# Autodesk Inventor assembly: Crossbrace
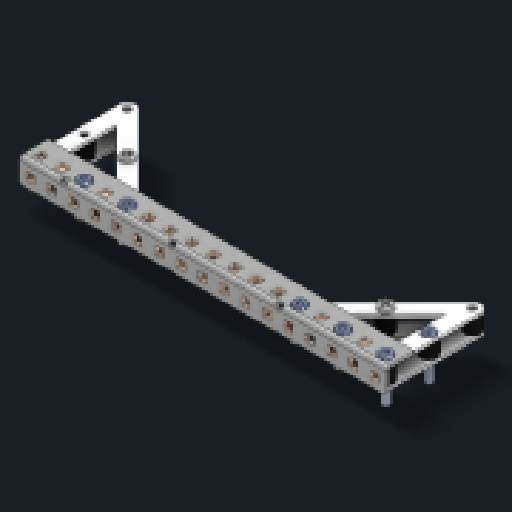
[picture p0: Inventor's stored thumbnail of the model, 512x512]
Saved by Autodesk Inventor 2025.1 (Build 291241000, 241)
## iProperties
Created: 2024-11-17
Part Number: Crossbrace
Document SubType Name: Assembly
Designer: avere
Author: avere
## Documents named in this file (14)
- C:\Users\avere\VEX\High Stakes\CAD\V3\Intake\Floating Stage\Crossbrace.iam
- C:\Users\avere\VEX\High Stakes\CAD\ROBOPROS-CAD-Inventor\Structure\C Channel\Aluminum 1x3x1 Half Thick Cut\Alu C Half Thick 1x3x1x17.ipt
- C:\Users\avere\VEX\High Stakes\CAD\V3\Intake\Floating Stage\Custom Parts\Arm Triangle Gusset.ipt
- C:\Users\avere\VEX\High Stakes\CAD\ROBOPROS-CAD-Inventor\Motion\Spacers\Spacer Nylon .375 OD.ipt
- C:\Users\avere\VEX\High Stakes\CAD\ROBOPROS-CAD-Inventor\Motion\Spacers\Spacer Nylon .375 OD\NSpacer .375 OD x .375.ipt
- C:\Users\avere\VEX\High Stakes\CAD\ROBOPROS-CAD-Inventor\Structure\Hardware\Screw Nylon - Pan Head\NScrew Pan Head Threaded .625.ipt
- C:\Users\avere\VEX\High Stakes\CAD\ROBOPROS-CAD-Inventor\Structure\Hardware\Screw Steel - Star.ipt
- C:\Users\avere\VEX\High Stakes\CAD\ROBOPROS-CAD-Inventor\Structure\Hardware\Nut Nylon\Nut Nylon - White.ipt
- C:\Users\avere\VEX\High Stakes\CAD\ROBOPROS-CAD-Inventor\Structure\Hardware\Nut Nylon.ipt
- C:\Users\avere\VEX\High Stakes\CAD\ROBOPROS-CAD-Inventor\Structure\Hardware\Screw Steel - Star\SScrew Star Smooth .750.ipt
- C:\Users\avere\VEX\High Stakes\CAD\ROBOPROS-CAD-Inventor\Motion\Shaft LS\LS Pillow Bearing Block.ipt
- C:\Users\avere\VEX\High Stakes\CAD\ROBOPROS-CAD-Inventor\Motion\Spacers\Washer Steel\SWasher .500 OD x .062500\SWasher .500 OD x .062500.ipt
- C:\Users\avere\VEX\High Stakes\CAD\ROBOPROS-CAD-Inventor\Motion\Spacers\Washer Steel\SWasher .500 OD x .062500.ipt
- C:\Users\avere\VEX\High Stakes\CAD\ROBOPROS-CAD-Inventor\Structure\Hardware\Screw Steel - Star\SScrew Star Smooth 1.250.ipt
## Components (37 placed, 9 different names)
1. Arm Triangle Gusset:1 — Insert:55, Mate:7, Mate:9, Insert:71, Insert:75, Insert:77, Insert:93, Insert:105
2. Arm Triangle Gusset:2 — Insert:55, Mate:7, Insert:72, Insert:73, Insert:74, Insert:76, Insert:94, Insert:102, Insert:103
3. Alu C Half Thick 1x3x1x17:1 — Mate:9, Insert:71, Insert:85, Mate:11, Insert:96, Insert:97, Insert:98, Insert:99, Insert:104, Insert:111
4. NSpacer .375 OD x .375:1 — Insert:73, Mate:12
5. NSpacer .375 OD x .375:2 — Insert:76
6. NSpacer .375 OD x .375:3 — Insert:77
7. NSpacer .375 OD x .375:4 — Insert:75
8. NSpacer .375 OD x .375:5 — Insert:74
9. NSpacer .375 OD x .375:6 — Insert:72
10. Arm Triangle Gusset:3 — Insert:95, Insert:100, Insert:101
11. Arm Triangle Gusset:4 — Insert:85, Insert:92, Mate:13
12. NSpacer .375 OD x .375:7
13. NSpacer .375 OD x .375:8
14. NSpacer .375 OD x .375:9
15. NSpacer .375 OD x .375:10
16. NSpacer .375 OD x .375:11
17. NSpacer .375 OD x .375:12 — Mate:11
18. NScrew Pan Head Threaded .625:1 — Insert:92
19. NScrew Pan Head Threaded .625:2 — Insert:93
20. Nut Nylon - White:1 — Insert:95
21. Nut Nylon - White:2 — Insert:94
22. SScrew Star Smooth .750:5 — Insert:96
23. SScrew Star Smooth .750:6 — Insert:97
24. SScrew Star Smooth .750:7 — Insert:98
25. SScrew Star Smooth .750:8 — Insert:99
26. Nut Nylon - White:3 — Insert:101
27. Nut Nylon - White:4 — Insert:100
28. Nut Nylon - White:5 — Insert:103
29. Nut Nylon - White:6 — Insert:102
30. LS Pillow Bearing Block:1 — Insert:104, Mate:12, Insert:106, Insert:107
31. SWasher .500 OD x .062500:1 — Insert:105
32. SScrew Star Smooth 1.250:9 — Insert:106
33. SScrew Star Smooth 1.250:10 — Insert:107
34. LS Pillow Bearing Block:2 — Insert:110, Insert:111
35. SScrew Star Smooth 1.250:11
36. SScrew Star Smooth 1.250:12
37. SWasher .500 OD x .062500:2 — Insert:110, Mate:13
## Relationships (42: Insert 36, Mate 6)
- Insert:55 (9.525 mm): Arm Triangle Gusset:1 ↔ Arm Triangle Gusset:2
- Mate:7: Arm Triangle Gusset:1 ↔ Arm Triangle Gusset:2
- Mate:9: Arm Triangle Gusset:1 ↔ Alu C Half Thick 1x3x1x17:1
- Insert:71: Arm Triangle Gusset:1 ↔ Alu C Half Thick 1x3x1x17:1
- Insert:72: Arm Triangle Gusset:2 ↔ NSpacer .375 OD x .375:6
- Insert:73: Arm Triangle Gusset:2 ↔ NSpacer .375 OD x .375:1
- Insert:74: Arm Triangle Gusset:2 ↔ NSpacer .375 OD x .375:5
- Insert:75: Arm Triangle Gusset:1 ↔ NSpacer .375 OD x .375:4
- Insert:76: Arm Triangle Gusset:2 ↔ NSpacer .375 OD x .375:2
- Insert:77: Arm Triangle Gusset:1 ↔ NSpacer .375 OD x .375:3
- [Insert] (9.525 mm): Arm Triangle Gusset:3 ↔ Arm Triangle Gusset:4
- [Mate]: Arm Triangle Gusset:3 ↔ Arm Triangle Gusset:4
- [Insert]: Arm Triangle Gusset:4 ↔ NSpacer .375 OD x .375:12
- [Insert]: Arm Triangle Gusset:4 ↔ NSpacer .375 OD x .375:7
- [Insert]: Arm Triangle Gusset:4 ↔ NSpacer .375 OD x .375:11
- [Insert]: Arm Triangle Gusset:3 ↔ NSpacer .375 OD x .375:10
- [Insert]: Arm Triangle Gusset:4 ↔ NSpacer .375 OD x .375:8
- [Insert]: Arm Triangle Gusset:3 ↔ NSpacer .375 OD x .375:9
- Insert:85: Alu C Half Thick 1x3x1x17:1 ↔ Arm Triangle Gusset:4
- Mate:11: Alu C Half Thick 1x3x1x17:1 ↔ NSpacer .375 OD x .375:12
- Insert:92: Arm Triangle Gusset:4 ↔ NScrew Pan Head Threaded .625:1
- Insert:93: Arm Triangle Gusset:1 ↔ NScrew Pan Head Threaded .625:2
- Insert:94: Arm Triangle Gusset:2 ↔ Nut Nylon - White:2
- Insert:95: Arm Triangle Gusset:3 ↔ Nut Nylon - White:1
- Insert:96: Alu C Half Thick 1x3x1x17:1 ↔ SScrew Star Smooth .750:5
- Insert:97: Alu C Half Thick 1x3x1x17:1 ↔ SScrew Star Smooth .750:6
- Insert:98: Alu C Half Thick 1x3x1x17:1 ↔ SScrew Star Smooth .750:7
- Insert:99: Alu C Half Thick 1x3x1x17:1 ↔ SScrew Star Smooth .750:8
- Insert:100: Arm Triangle Gusset:3 ↔ Nut Nylon - White:4
- Insert:101: Arm Triangle Gusset:3 ↔ Nut Nylon - White:3
- Insert:102: Arm Triangle Gusset:2 ↔ Nut Nylon - White:6
- Insert:103: Arm Triangle Gusset:2 ↔ Nut Nylon - White:5
- Insert:104: Alu C Half Thick 1x3x1x17:1 ↔ LS Pillow Bearing Block:1
- Mate:12: NSpacer .375 OD x .375:1 ↔ LS Pillow Bearing Block:1
- Insert:105: Arm Triangle Gusset:1 ↔ SWasher .500 OD x .062500:1
- Insert:106: LS Pillow Bearing Block:1 ↔ SScrew Star Smooth 1.250:9
- Insert:107: LS Pillow Bearing Block:1 ↔ SScrew Star Smooth 1.250:10
- [Insert]: LS Pillow Bearing Block:2 ↔ SScrew Star Smooth 1.250:11
- [Insert]: LS Pillow Bearing Block:2 ↔ SScrew Star Smooth 1.250:12
- Insert:110: LS Pillow Bearing Block:2 ↔ SWasher .500 OD x .062500:2
- Insert:111: Alu C Half Thick 1x3x1x17:1 ↔ LS Pillow Bearing Block:2
- Mate:13: Arm Triangle Gusset:4 ↔ SWasher .500 OD x .062500:2
## Named parameters: d94_d60 = 9.525 mm, d95_d61 = 0 mm, d96_d88 = 0 mm, d97_d89 = 0 mm, d98_d90 = 0 mm, d99_d91 = 0 mm, d100_d92 = 0 mm, d101_d93 = 0 mm, d134_d132 = 0 mm, d135_d133 = 0 mm
